# Autodesk Inventor assembly: POJAZD
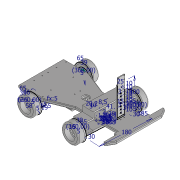
[picture p0: Inventor's stored thumbnail of the model, 180x180]
Saved by Autodesk Inventor 2020 (Build 240168000, 168)
## iProperties
Created: 2020-03-14
Part Number: POJAZD
Document SubType Name: Assembly
Designer: JakubTomaszewski
Author: JakubTomaszewski
## Documents named in this file (14)
- C:\Users\JakubTomaszewski\Documents\Inventor\Autonomiczny Robot - TOFIC\POJAZD.iam
- C:\Users\JakubTomaszewski\Documents\Inventor\Autonomiczny Robot - TOFIC\Podwozie.ipt
- C:\Users\JakubTomaszewski\Documents\Inventor\Autonomiczny Robot - TOFIC\Serwo.ipt
- C:\Users\JakubTomaszewski\Documents\Inventor\Autonomiczny Robot - TOFIC\Manipulator.ipt
- C:\Users\JakubTomaszewski\Documents\Inventor\Autonomiczny Robot - TOFIC\Rama_1.ipt
- C:\Users\JakubTomaszewski\Documents\Inventor\Autonomiczny Robot - TOFIC\Rama_2.ipt
- C:\Users\JakubTomaszewski\Documents\Inventor\Autonomiczny Robot - TOFIC\KOŁO.ipt
- C:\Users\JakubTomaszewski\Documents\Inventor\Autonomiczny Robot - TOFIC\ObudowaSilnika.ipt
- C:\Users\JakubTomaszewski\Documents\Inventor\Autonomiczny Robot - TOFIC\ObudowaSilnika2.ipt
- C:\Users\JakubTomaszewski\Documents\Inventor\Autonomiczny Robot - TOFIC\Silnik.ipt
- C:\Users\JakubTomaszewski\Documents\Inventor\Autonomiczny Robot - TOFIC\Silnik2.ipt
- C:\Users\JakubTomaszewski\Documents\Inventor\Autonomiczny Robot - TOFIC\Kamerka-Stojak.ipt
- C:\Users\JakubTomaszewski\Documents\Inventor\Autonomiczny Robot - TOFIC\Kamerka-Mocowanie.ipt
- C:\Users\JakubTomaszewski\Documents\Inventor\Autonomiczny Robot - TOFIC\Bateria-uchwyt.ipt
## Components (19 placed, 13 different names)
1. Podwozie:1 — SERWO, Sztywne:4, Sztywne:5, Kamerak-Stojak, Sztywne:12, Sztywne:13, Sztywne:14, Sztywne:15
2. Serwo:1 — SERWO, Wstawiające:6
3. Manipulator:1 — Wstawiające:6, Sztywne:17
4. Rama_2:1 — Wstawiające:9, Wstawiające:11, Sztywne:18
5. KOŁO:1 — Wstawiające:11
6. KOŁO:2 — Wstawiające:9
7. ObudowaSilnika:1 — Sztywne:4, Sztywne:6
8. ObudowaSilnika2:1 — Sztywne:5, Sztywne:16
9. Silnik:1 — Sztywne:6, Wstawiające:10
10. KOŁO:3 — Wstawiające:7
11. KOŁO:4 — Wstawiające:10
12. Kamerka-Stojak:1 — Kamerak-Stojak, Sztywne:11
13. Kamerka-Mocowanie:1 — Sztywne:11
14. Bateria-uchwyt:1 — Sztywne:14
15. Bateria-uchwyt:2 — Sztywne:15
16. Bateria-uchwyt:3 — Sztywne:12
17. Bateria-uchwyt:4 — Sztywne:13
18. Silnik2:2 — Sztywne:16, Wstawiające:7
19. Rama_1:1 — Sztywne:17, Sztywne:18
## Relationships (18: WeldJoint 13, Insert 5)
- SERWO [WeldJoint]: Podwozie:1 ↔ Serwo:1
- Sztywne:4 [WeldJoint]: Podwozie:1 ↔ ObudowaSilnika:1
- Sztywne:5 [WeldJoint]: Podwozie:1 ↔ ObudowaSilnika2:1
- Sztywne:6 [WeldJoint]: ObudowaSilnika:1 ↔ Silnik:1
- Wstawiające:6 [Insert] (-5 mm): Serwo:1 ↔ Manipulator:1
- Kamerak-Stojak [WeldJoint]: Podwozie:1 ↔ Kamerka-Stojak:1
- Sztywne:11 [WeldJoint]: Kamerka-Stojak:1 ↔ Kamerka-Mocowanie:1
- Sztywne:12 [WeldJoint]: Podwozie:1 ↔ Bateria-uchwyt:3
- Sztywne:13 [WeldJoint]: Podwozie:1 ↔ Bateria-uchwyt:4
- Sztywne:14 [WeldJoint]: Podwozie:1 ↔ Bateria-uchwyt:1
- Sztywne:15 [WeldJoint]: Podwozie:1 ↔ Bateria-uchwyt:2
- Sztywne:16 [WeldJoint]: ObudowaSilnika2:1 ↔ Silnik2:2
- Wstawiające:7 [Insert] (-5 mm): KOŁO:3 ↔ Silnik2:2
- Wstawiające:9 [Insert] (-5 mm): Rama_2:1 ↔ KOŁO:2
- Wstawiające:10 [Insert] (-5 mm): Silnik:1 ↔ KOŁO:4
- Wstawiające:11 [Insert] (-5 mm): Rama_2:1 ↔ KOŁO:1
- Sztywne:17 [WeldJoint]: Manipulator:1 ↔ Rama_1:1
- Sztywne:18 [WeldJoint]: Rama_2:1 ↔ Rama_1:1
